# Autodesk Inventor assembly: assembled
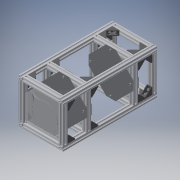
[picture p0: Inventor's stored thumbnail of the model, 180x180]
Saved by Autodesk Inventor 2016 (Build 200138000, 138)
## iProperties
Created: 2016-07-21
Part Number: assembled
Document SubType Name: Assembly
Designer: Jonathan
Author: Jonathan
## Documents named in this file (5)
- C:\Users\Jonathan\Desktop\Models\Three Panel Detector\assembled.iam
- C:\Users\Jonathan\Desktop\Models\Three Panel Detector\frame\frame.iam
- C:\Users\Jonathan\Desktop\Models\Three Panel Detector\frame\separator\assembled cover.iam
- C:\Users\Jonathan\Desktop\Models\Three Panel Detector\panel\loopPanel.iam
- C:\Users\Jonathan\Desktop\Models\Three Panel Detector\frameSpecifications.xlsx
## Components (9 placed, 3 different names)
1. frame:1 [sub-assembly] — Mate:1, Mate:2, Mate:3, Flush:5, Flush:6, Mate:8, Mate:9, Flush:15, Flush:16, Angle:1
2. assembled cover:1 [sub-assembly] — Mate:2, Flush:1, Flush:2, Flush:3, Flush:4, Mate:17
3. assembled cover:2 [sub-assembly] — Mate:1, Flush:1, Flush:4, Flush:5, Flush:6, Mate:16
4. assembled cover:3 [sub-assembly] — Mate:3, Flush:2, Flush:3, Mate:18, Mate:19
5. loopPanel:2 [sub-assembly] — Flush:21, Flush:22, Mate:17, Mate:19
6. loopPanel:3 [sub-assembly] — Flush:20, Flush:21, Flush:22, Flush:23, Mate:18, Angle:1
7. loopPanel:4 [sub-assembly] — Flush:20, Flush:23, Mate:16
8. assembled cover:5 [sub-assembly] — Flush:12, Flush:13, Mate:8, Flush:15, Flush:16
9. assembled cover:6 [sub-assembly] — Flush:12, Flush:13, Mate:9
## Relationships (24: Flush 14, Mate 9, Angle 1)
- Mate:1: frame:1 ↔ assembled cover:2
- Mate:2: frame:1 ↔ assembled cover:1
- Mate:3: frame:1 ↔ assembled cover:3
- Flush:1: assembled cover:1 ↔ assembled cover:2
- Flush:2: assembled cover:1 ↔ assembled cover:3
- Flush:3: assembled cover:1 ↔ assembled cover:3
- Flush:4: assembled cover:1 ↔ assembled cover:2
- Flush:5: frame:1 ↔ assembled cover:2
- Flush:6: frame:1 ↔ assembled cover:2
- Flush:12: assembled cover:5 ↔ assembled cover:6
- Flush:13: assembled cover:5 ↔ assembled cover:6
- Mate:8: frame:1 ↔ assembled cover:5
- Mate:9: frame:1 ↔ assembled cover:6
- Flush:15: frame:1 ↔ assembled cover:5
- Flush:16: frame:1 ↔ assembled cover:5
- Flush:20: loopPanel:3 ↔ loopPanel:4
- Flush:21: loopPanel:2 ↔ loopPanel:3
- Flush:22: loopPanel:2 ↔ loopPanel:3
- Flush:23: loopPanel:3 ↔ loopPanel:4
- Mate:16: assembled cover:2 ↔ loopPanel:4
- Mate:17: assembled cover:1 ↔ loopPanel:2
- Mate:18: assembled cover:3 ↔ loopPanel:3
- Mate:19: assembled cover:3 ↔ loopPanel:2
- Angle:1 (0 deg): frame:1 ↔ loopPanel:3
## Named parameters: height = 400 mm, width = 150 mm, topSeparation = 100 mm, botSeparation = 200 mm, panelChamfer = 75 mm
